# Autodesk Inventor assembly: Frame_Welded
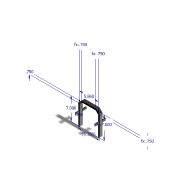
[picture p0: Inventor's stored thumbnail of the model, 180x180]
Saved by Autodesk Inventor 2020 (Build 240168000, 168)
## iProperties
Created: 2019-05-22
Part Number: Frame_Welded
Document SubType Name: Weldment
Designer: chitl
Weld Material: Steel, Mild, Welded
_SolveAssemblyDoc: Frame Generator Solve Assembly
_Version: 15.0.0
Author: chitl
## Documents named in this file (4)
- C:\Users\chitl\Desktop\OneWheel\Wheel Assembled\Chassis\Handle_Frame\Frame_Welded.iam
- C:\Users\chitl\Desktop\OneWheel\Wheel Assembled\Chassis\Handle_Frame\Handle_Frame.ipt
- C:\Users\chitl\Desktop\OneWheel\Wheel Assembled\Chassis\Handle_Frame\Frame_Welded\Frame\Frame 1558516499646.iam
- C:\Users\chitl\Desktop\OneWheel\Wheel Assembled\Chassis\Handle_Frame\Cover_attachment.ipt
## Components (6 placed, 3 different names)
1. Handle_Frame:1
2. Frame 1558516499646:1 [sub-assembly] — Mate:1, Mate:2, Mate:3, Mate:4, Mate:6, Mate:7, Mate:9
3. Cover_attachment:1 — Mate:1, Mate:4, Mate:5
4. Cover_attachment:2 — Mate:2, Mate:3, Mate:5
5. Cover_attachment:3 — Mate:6, Mate:8, Mate:9
6. Cover_attachment:4 — Mate:7, Mate:8
## Relationships (9: Mate 9)
- Mate:1: Frame 1558516499646:1 ↔ Cover_attachment:1
- Mate:2: Frame 1558516499646:1 ↔ Cover_attachment:2
- Mate:3: Frame 1558516499646:1 ↔ Cover_attachment:2
- Mate:4: Frame 1558516499646:1 ↔ Cover_attachment:1
- Mate:5: Cover_attachment:1 ↔ Cover_attachment:2
- Mate:6: Frame 1558516499646:1 ↔ Cover_attachment:3
- Mate:7: Frame 1558516499646:1 ↔ Cover_attachment:4
- Mate:8: Cover_attachment:3 ↔ Cover_attachment:4
- Mate:9: Frame 1558516499646:1 ↔ Cover_attachment:3
